# Autodesk Inventor assembly: Spool Assembly
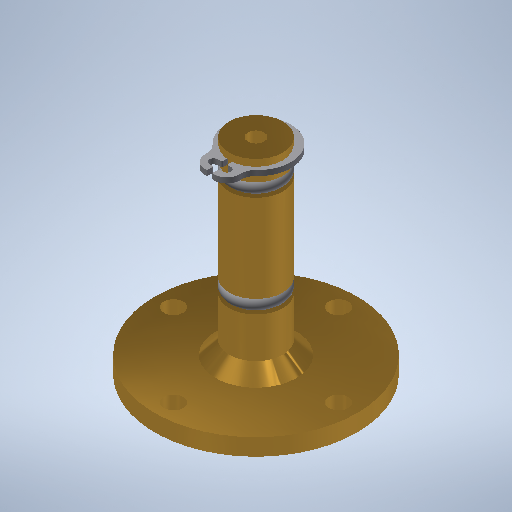
[picture p0: Inventor's stored thumbnail of the model, 512x512]
Saved by Autodesk Inventor 2025 (Build 290162000, 162)
## iProperties
Created: 2021-01-08
Part Number: Spool Assembly
Document SubType Name: Assembly
Designer: caleb
Author: caleb
## Documents named in this file (4)
- C:\Users\cfang\Desktop\nebraska-silicon-lab\Hardware\ETL\Module Assembly\Picker Tool\Spool Assembly.iam
- C:\Users\cfang\Desktop\nebraska-silicon-lab\Hardware\ETL\Module Assembly\Picker Tool\Picker Spool.ipt
- C:\Users\cfang\Desktop\nebraska-silicon-lab\Hardware\ETL\Module Assembly\Picker Tool\9452K160_OIL-RESISTANT BUNA-N MULTIPURPOSE O-RING.ipt
- C:\Users\cfang\Desktop\nebraska-silicon-lab\Hardware\ETL\Module Assembly\Picker Tool - V2\98541A116_External Retaining Ring\98541A116_External Retaining Ring.ipt
## Components (5 placed, 3 different names)
1. Picker Spool:1 — Rigid:1, Rigid:2, Rigid:3, Insert:1
2. 9452K160_OIL-RESISTANT BUNA-N MULTIPURPOSE O-RING:1 — Rigid:1
3. 9452K160_OIL-RESISTANT BUNA-N MULTIPURPOSE O-RING:2 — Rigid:2
4. 9452K160_OIL-RESISTANT BUNA-N MULTIPURPOSE O-RING:3 — Rigid:3
5. 98541A116_External Retaining Ring:1 — Insert:1
## Relationships (4: WeldJoint 3, Insert 1)
- Rigid:1 [WeldJoint]: Picker Spool:1 ↔ 9452K160_OIL-RESISTANT BUNA-N MULTIPURPOSE O-RING:1
- Rigid:2 [WeldJoint]: Picker Spool:1 ↔ 9452K160_OIL-RESISTANT BUNA-N MULTIPURPOSE O-RING:2
- Rigid:3 [WeldJoint] (-0.508 mm): Picker Spool:1 ↔ 9452K160_OIL-RESISTANT BUNA-N MULTIPURPOSE O-RING:3
- Insert:1: Picker Spool:1 ↔ 98541A116_External Retaining Ring:1
